# Autodesk Inventor assembly: Leg_Loadpipe_Connector
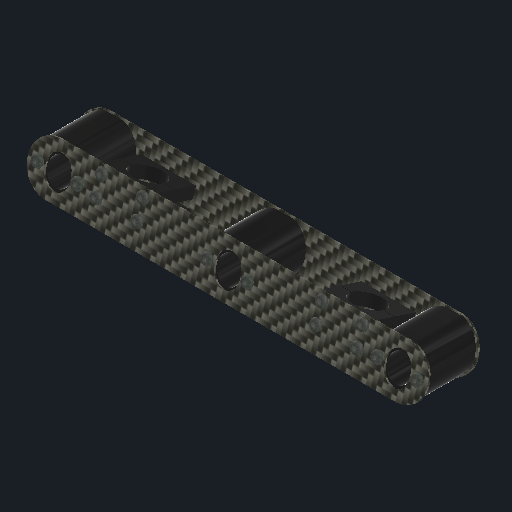
[picture p0: Inventor's stored thumbnail of the model, 512x512]
Saved by Autodesk Inventor 2024.1 (Build 281209000, 209)
## iProperties
Created: 2023-06-08
Part Number: Leg_Loadpipe_Connector
Document SubType Name: Assembly
Designer: dzw04
Author: dzw04
## Documents named in this file (6)
- C:\Users\dzw04\Saxion\Mechatronica Lectoraat LMECH LED - Database ARG\Component_Database\SARAX\01. CAD\01. 3D_Drawing\02. Sub_Assemblies\Landing_Gear\02. Sub_Assemblies\Leg_Loadpipe_Connector.iam
- C:\Users\dzw04\Saxion\Mechatronica Lectoraat LMECH LED - Database ARG\Component_Database\SARAX\01. CAD\01. 3D_Drawing\02. Sub_Assemblies\Landing_Gear\01. Parts\Leg_Loadpipe_Plate_Inner.ipt
- C:\Users\dzw04\Saxion\Mechatronica Lectoraat LMECH LED - Database ARG\Component_Database\SARAX\01. CAD\01. 3D_Drawing\02. Sub_Assemblies\Landing_Gear\02. Sub_Assemblies\Leg_Loadpipe_Mount.iam
- C:\Users\dzw04\OneDrive - Saxion\Documenten\Inventor\Content Center Files\R2024\en-US\ISO 7380-1\ISO 7380-1 - M3 x 6.ipt
- C:\Users\dzw04\Saxion\Mechatronica Lectoraat LMECH LED - Database ARG\Component_Database\SARAX\01. CAD\01. 3D_Drawing\02. Sub_Assemblies\Landing_Gear\01. Parts\Leg_Loadpipe_Plate_Outer.ipt
- C:\Users\dzw04\Saxion\Mechatronica Lectoraat LMECH LED - Database ARG\Component_Database\SARAX\01. CAD\01. 3D_Drawing\02. Sub_Assemblies\Landing_Gear\02. Sub_Assemblies\16mm_Tube_Connector.iam
## Components (21 placed, 5 different names)
1. Leg_Loadpipe_Plate_Inner:1 — Mate:2, Mate:3, Mate:4, Mate:5, Insert:1, Insert:2, Mate:8, Mate:9, Mate:10
2. Leg_Loadpipe_Plate_Outer:1 — Mate:5, Mate:6, Mate:7, Insert:3, Insert:4
3. ISO 7380-1 M3 x 6:1 — Insert:1
4. ISO 7380-1 M3 x 6:2 — Insert:2
5. ISO 7380-1 M3 x 6:3 — Insert:3
6. ISO 7380-1 M3 x 6:4 — Insert:4
7. Leg_Loadpipe_Mount:1 [sub-assembly] — Mate:2, Mate:3, Mate:4, Mate:6, Mate:7
8. ISO 7380-1 M3 x 6:5
9. ISO 7380-1 M3 x 6:6
10. ISO 7380-1 M3 x 6:7
11. ISO 7380-1 M3 x 6:8
12. Leg_Loadpipe_Mount:2 [sub-assembly]
13. ISO 7380-1 M3 x 6:9
14. ISO 7380-1 M3 x 6:10
15. ISO 7380-1 M3 x 6:11
16. ISO 7380-1 M3 x 6:12
17. Leg_Loadpipe_Mount:3 [sub-assembly]
18. 16mm_Tube_Connector:1 [sub-assembly] — Mate:8, Mate:9, Mate:10
19. 16mm_Tube_Connector:2 [sub-assembly]
20. 16mm_Tube_Connector:3 [sub-assembly]
21. 16mm_Tube_Connector:4 [sub-assembly]
## Component patterns: (3 elements, first: ISO 7380-1 M3 x 6:1 + ISO 7380-1 M3 x 6:2 + ISO 7380-1 M3 x 6:3 + ISO 7380-1 M3 x 6:4 + Leg_Loadpipe_Mount:1), (4 elements, first: 16mm_Tube_Connector:1)
## Relationships (13: Mate 9, Insert 4)
- Mate:2: Leg_Loadpipe_Plate_Inner:1 ↔ Leg_Loadpipe_Mount:1
- Mate:3: Leg_Loadpipe_Plate_Inner:1 ↔ Leg_Loadpipe_Mount:1
- Mate:4: Leg_Loadpipe_Plate_Inner:1 ↔ Leg_Loadpipe_Mount:1
- Mate:5 (22.5 mm): Leg_Loadpipe_Plate_Inner:1 ↔ Leg_Loadpipe_Plate_Outer:1
- Mate:6: Leg_Loadpipe_Plate_Outer:1 ↔ Leg_Loadpipe_Mount:1
- Mate:7: Leg_Loadpipe_Plate_Outer:1 ↔ Leg_Loadpipe_Mount:1
- Insert:1: Leg_Loadpipe_Plate_Inner:1 ↔ ISO 7380-1 M3 x 6:1
- Insert:2: Leg_Loadpipe_Plate_Inner:1 ↔ ISO 7380-1 M3 x 6:2
- Insert:3: Leg_Loadpipe_Plate_Outer:1 ↔ ISO 7380-1 M3 x 6:3
- Insert:4: Leg_Loadpipe_Plate_Outer:1 ↔ ISO 7380-1 M3 x 6:4
- Mate:8: Leg_Loadpipe_Plate_Inner:1 ↔ 16mm_Tube_Connector:1
- Mate:9: Leg_Loadpipe_Plate_Inner:1 ↔ 16mm_Tube_Connector:1
- Mate:10: Leg_Loadpipe_Plate_Inner:1 ↔ 16mm_Tube_Connector:1
